# Autodesk Inventor assembly: Assembly_Trial_1
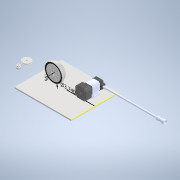
[picture p0: Inventor's stored thumbnail of the model, 180x180]
Saved by Autodesk Inventor 2022 (Build 260153000, 153)
## iProperties
Created: 2022-01-01
Part Number: Assembly_Trial_1
Document SubType Name: Assembly
Designer: Mlees
Author: Mlees
## Documents named in this file (13)
- E:\404 Engineering Arm\Assembly_Trial_1.iam
- E:\404 Engineering Arm\Downloaded Parts\Nema17-115oz-in-holding\stp-mtr-17060w.ipt
- E:\404 Engineering Arm\Downloaded Parts\nema-17-motor-mount-1.snapshot.1\NEMA_17_Bracket.ipt
- E:\404 Engineering Arm\Downloaded Parts\nema17-speed-reducer-1.snapshot.9\24_Teeth_Sun_Gear.step.ipt
- E:\404 Engineering Arm\Downloaded Parts\nema17-speed-reducer-1.snapshot.9\36_Teeth_Planet_Gear.step.ipt
- E:\404 Engineering Arm\Downloaded Parts\nema17-speed-reducer-1.snapshot.9\96_Teeth_Gear.step.ipt
- E:\404 Engineering Arm\Downloaded Parts\nema17-speed-reducer-1.snapshot.9\Gear_Cover.ipt
- E:\404 Engineering Arm\Downloaded Parts\nema17-speed-reducer-1.snapshot.9\Plamet_Carrier.ipt
- E:\404 Engineering Arm\Created Parts\Base.ipt
- E:\404 Engineering Arm\Downloaded Parts\Pully_System\GT2 20T Drive Pulley.ipt
- E:\404 Engineering Arm\Downloaded Parts\Pully_System\GT2 60T Drive Pulley.ipt
- E:\404 Engineering Arm\Downloaded Parts\75mm_Harmonic_Drive\HarmonicDrive75mmV2.iam
- E:\404 Engineering Arm\Downloaded Parts\75mm_Harmonic_Drive\Radial Bearings\6815 bearing.ipt
## Components (14 placed, 12 different names)
1. stp-mtr-17060w:1 — Rigid:1, Rotational:1
2. NEMA_17_Bracket:1 — Rigid:1, Rigid:2, Rigid:4
3. 24_Teeth_Sun_Gear.step:1 — Rotational:1, Flush:1, Mate:1, Mate:2, Mate:3, Flush:4, Flush:5
4. 36_Teeth_Planet_Gear.step:1 — Mate:3, Flush:5, Mate:5
5. 96_Teeth_Gear.step:1 — Rigid:2, Rigid:3
6. Gear_Cover:1 — Rigid:3
7. Plamet_Carrier:1 — Mate:4, Mate:5, Mate:6
8. 36_Teeth_Planet_Gear.step:2 — Flush:1, Mate:1, Mate:6
9. 36_Teeth_Planet_Gear.step:3 — Mate:2, Flush:4, Mate:4
10. Base:1 — Rigid:4
11. GT2 20T Drive Pulley:1
12. GT2 60T Drive Pulley:1
13. HarmonicDrive75mmV2:1 [sub-assembly]
14. 6815 bearing:1
## Relationships (14: Mate 6, WeldJoint 4, Flush 3, RevoluteJoint 1)
- Rigid:1 [WeldJoint]: stp-mtr-17060w:1 ↔ NEMA_17_Bracket:1
- Rigid:2 [WeldJoint]: NEMA_17_Bracket:1 ↔ 96_Teeth_Gear.step:1
- Rotational:1 [RevoluteJoint]: stp-mtr-17060w:1 ↔ 24_Teeth_Sun_Gear.step:1
- Flush:1: 24_Teeth_Sun_Gear.step:1 ↔ 36_Teeth_Planet_Gear.step:2
- Mate:1 (14.986 mm): 24_Teeth_Sun_Gear.step:1 ↔ 36_Teeth_Planet_Gear.step:2
- Mate:2 (14.986 mm): 24_Teeth_Sun_Gear.step:1 ↔ 36_Teeth_Planet_Gear.step:3
- Mate:3 (14.986 mm): 24_Teeth_Sun_Gear.step:1 ↔ 36_Teeth_Planet_Gear.step:1
- Flush:4: 24_Teeth_Sun_Gear.step:1 ↔ 36_Teeth_Planet_Gear.step:3
- Flush:5: 24_Teeth_Sun_Gear.step:1 ↔ 36_Teeth_Planet_Gear.step:1
- Mate:4: Plamet_Carrier:1 ↔ 36_Teeth_Planet_Gear.step:3
- Mate:5: 36_Teeth_Planet_Gear.step:1 ↔ Plamet_Carrier:1
- Mate:6: Plamet_Carrier:1 ↔ 36_Teeth_Planet_Gear.step:2
- Rigid:3 [WeldJoint]: 96_Teeth_Gear.step:1 ↔ Gear_Cover:1
- Rigid:4 [WeldJoint]: NEMA_17_Bracket:1 ↔ Base:1
